# Autodesk Inventor assembly: brush holder assy
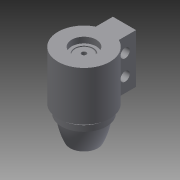
[picture p0: Inventor's stored thumbnail of the model, 180x180]
Saved by Autodesk Inventor 2013 SP2 (Build 170200200, 200)
## iProperties
Created: 2017-08-28
Part Number: brush holder assy
Document SubType Name: Assembly
Designer: hdv
Author: hdv
## Documents named in this file (4)
- C:\Users\hdv\Dropbox\Projects\Inventor\PaintBot_3\Brush holder\brush holder assy.iam
- C:\Users\hdv\Dropbox\Projects\Inventor\PaintBot_3\Brush holder\brush holder.ipt
- C:\Users\hdv\Dropbox\Projects\Inventor\PaintBot_3\Brush holder\brush fitting parta.ipt
- C:\Users\hdv\Dropbox\Projects\Inventor\PaintBot_3\Brush holder\brush fitting partb.ipt
## Components (3 placed, 3 different names)
1. brush holder:1 — Mate:1
2. brush fitting parta:1 — Mate:1, Mate:3, Mate:4
3. brush fitting partb:1 — Mate:3, Mate:4
## Relationships (3: Mate 3)
- Mate:1: brush holder:1 ↔ brush fitting parta:1
- Mate:3: brush fitting parta:1 ↔ brush fitting partb:1
- Mate:4: brush fitting parta:1 ↔ brush fitting partb:1
